# Autodesk Inventor assembly: Eierkocher_final
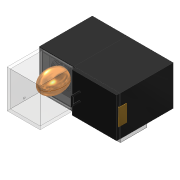
[picture p0: Inventor's stored thumbnail of the model, 180x180]
Saved by Autodesk Inventor 2020 (Build 240168000, 168)
## iProperties
Created: 2022-02-08
Part Number: Eierkocher_final
Document SubType Name: Assembly
Designer: Julian Uhl
Author: Julian Uhl
## Documents named in this file (33)
- C:\Schule\Eier-Inventor\Eierkocher_final.iam
- C:\Schule\Eier-Inventor\Eierkocher_final.ipt
- C:\Schule\Eier-Inventor\EierkocherTeil2.ipt
- C:\Schule\Eier-Inventor\Eihalter_Halter.ipt
- C:\Schule\Eier-Inventor\Raspberry_Dummy.ipt
- C:\Schule\Eier-Inventor\Dichtung_final.ipt
- C:\Schule\Eier-Inventor\Deckel_Koch_final.ipt
- C:\Schule\Eier-Inventor\Eihalter.ipt
- C:\Schule\Eier-Inventor\Ei_groß.ipt
- C:\Schule\Eier-Inventor\Senso_Halter.ipt
- C:\Schule\Eier-Inventor\Display_Dummy.ipt
- C:\Schule\Eier-Inventor\Heiz_Dummy.ipt
- C:\Schule\Eier-Inventor\Wasserbecken.ipt
- C:\Schule\Eier-Inventor\DeckelMess_Better.ipt
- C:\Schule\Eier-Inventor\Schanier1.ipt
- C:\Schule\Eier-Inventor\Schanier2.ipt
- C:\Schule\Eier-Inventor\Schanier3.ipt
- C:\Schule\Eier-Inventor\Ei.ipt
- C:\Schule\Eier-Inventor\Sensor_Dummy.ipt
- C:\Schule\Eier-Inventor\Eierkocher_final\AIP\FEA\dvr005z6o.fins
- C:\Schule\Eier-Inventor\Eierkocher_final\AIP\FEA\dvr005z6o.fsat
- C:\Schule\Eier-Inventor\Eierkocher_final\AIP\FEA\dvr005z6o.ftes
- C:\Schule\Eier-Inventor\Eierkocher_final\AIP\FEA\dvr005z6o.fwiz
- C:\Schule\Eier-Inventor\Eierkocher_final\AIP\FEA\dvr005zeo.fmsh
- C:\Schule\Eier-Inventor\Eierkocher_final\AIP\FEA\dvr005zep.fres
- C:\Schule\Eier-Inventor\Eierkocher_final\AIP\FEA\dvuwvce80.fins
- C:\Schule\Eier-Inventor\Eierkocher_final\AIP\FEA\dvuwvce80.fsat
- C:\Schule\Eier-Inventor\Eierkocher_final\AIP\FEA\dvuwvce80.ftes
- C:\Schule\Eier-Inventor\Eierkocher_final\AIP\FEA\dvuwvce80.fwiz
- C:\Schule\Eier-Inventor\Eierkocher_final\AIP\FEA\dvuwvcekg.fmsh
- C:\Schule\Eier-Inventor\Eierkocher_final\AIP\FEA\dvuwvcekh.fres
- C:\Schule\Eier-Inventor\Eierkocher_final\AIP\FEA\dvyb0c0e8.fmsh
- C:\Schule\Eier-Inventor\Eierkocher_final\AIP\FEA\dvyb0c0e9.fres
## Components (21 placed, 18 different names)
1. Eierkocher_final:1 — Passend:1, Fluchtend:1, Fluchtend:2, Passend:2, Passend:3, Fluchtend:3, Passend:4, Passend:5, Fluchtend:4, Passend:6, Passend:7, Fluchtend:5, Passend:8, Passend:9, Fluchtend:6, Passend:13, Passend:14, Passend:15, Passend:17, Passend:18, Passend:35, Passend:36, Passend:37, Passend:41, Passend:44, Passend:54, Passend:55
2. EierkocherTeil2:1 — Passend:1, Fluchtend:1, Fluchtend:2, Passend:10, Passend:11, Passend:12, Passend:25, Passend:26, Passend:27, Passend:32, Fluchtend:9, Fluchtend:10, Passend:50, Fluchtend:13, Fluchtend:14
3. Eihalter_Halter:1 — Passend:2, Passend:3, Fluchtend:3
4. Eihalter_Halter:2 — Passend:4, Passend:5, Fluchtend:4
5. Eihalter_Halter:3 — Passend:6, Passend:7, Fluchtend:5
6. Eihalter_Halter:4 — Passend:8, Passend:9, Fluchtend:6, Passend:53
7. Raspberry_Dummy:1 — Passend:10, Passend:11, Passend:12
8. Dichtung_final:1 — Passend:13, Passend:14, Passend:15, Passend:16
9. Deckel_Koch_final:1 — Passend:16, Passend:17, Passend:18
10. Senso_Halter:1 — Passend:25, Passend:26, Passend:27, Passend:51, Passend:52, Passend:61, Passend:62, Passend:63
11. Display_Dummy:1 — Passend:32, Fluchtend:9, Fluchtend:10
12. Wasserbecken:1 — Passend:35, Passend:36, Passend:37, Passend:58, Passend:59, Passend:60
13. DeckelMess_Better:1 — Passend:47, Passend:48, Passend:49
14. Schanier1:1 — Passend:45, Fluchtend:11, Passend:47, Passend:48, Passend:49
15. Schanier2:1 — Passend:46, Fluchtend:12, Passend:50, Fluchtend:13, Fluchtend:14
16. Schanier3:1 — Passend:45, Fluchtend:11, Passend:46, Fluchtend:12
17. Ei:1 — Passend:51, Passend:52
18. Eihalter:1 — Passend:53, Passend:54, Passend:55, Passend:56, Passend:57
19. Ei_groß:1 — Passend:56, Passend:57
20. Heiz_Dummy:1 — Passend:58, Passend:59, Passend:60
21. Sensor_Dummy:1 — Passend:61, Passend:62, Passend:63
## Relationships (58: Mate 46, Flush 12)
- Passend:1 [Mate]: Eierkocher_final:1 ↔ EierkocherTeil2:1
- Fluchtend:1 [Flush]: Eierkocher_final:1 ↔ EierkocherTeil2:1
- Fluchtend:2 [Flush]: Eierkocher_final:1 ↔ EierkocherTeil2:1
- Passend:2 [Mate]: Eierkocher_final:1 ↔ Eihalter_Halter:1
- Passend:3 [Mate]: Eierkocher_final:1 ↔ Eihalter_Halter:1
- Fluchtend:3 [Flush] (25 mm): Eierkocher_final:1 ↔ Eihalter_Halter:1
- Passend:4 [Mate]: Eierkocher_final:1 ↔ Eihalter_Halter:2
- Passend:5 [Mate]: Eierkocher_final:1 ↔ Eihalter_Halter:2
- Fluchtend:4 [Flush] (25 mm): Eierkocher_final:1 ↔ Eihalter_Halter:2
- Passend:6 [Mate]: Eierkocher_final:1 ↔ Eihalter_Halter:3
- Passend:7 [Mate]: Eierkocher_final:1 ↔ Eihalter_Halter:3
- Fluchtend:5 [Flush] (25 mm): Eierkocher_final:1 ↔ Eihalter_Halter:3
- Passend:8 [Mate]: Eierkocher_final:1 ↔ Eihalter_Halter:4
- Passend:9 [Mate]: Eierkocher_final:1 ↔ Eihalter_Halter:4
- Fluchtend:6 [Flush] (25 mm): Eierkocher_final:1 ↔ Eihalter_Halter:4
- Passend:10 [Mate]: EierkocherTeil2:1 ↔ Raspberry_Dummy:1
- Passend:11 [Mate] (15 mm): EierkocherTeil2:1 ↔ Raspberry_Dummy:1
- Passend:12 [Mate] (20 mm): EierkocherTeil2:1 ↔ Raspberry_Dummy:1
- Passend:13 [Mate]: Eierkocher_final:1 ↔ Dichtung_final:1
- Passend:14 [Mate] (1 mm): Eierkocher_final:1 ↔ Dichtung_final:1
- Passend:15 [Mate] (1 mm): Eierkocher_final:1 ↔ Dichtung_final:1
- Passend:16 [Mate]: Dichtung_final:1 ↔ Deckel_Koch_final:1
- Passend:17 [Mate]: Eierkocher_final:1 ↔ Deckel_Koch_final:1
- Passend:18 [Mate]: Eierkocher_final:1 ↔ Deckel_Koch_final:1
- Passend:25 [Mate]: EierkocherTeil2:1 ↔ Senso_Halter:1
- Passend:26 [Mate]: EierkocherTeil2:1 ↔ Senso_Halter:1
- Passend:27 [Mate]: EierkocherTeil2:1 ↔ Senso_Halter:1
- Passend:32 [Mate]: EierkocherTeil2:1 ↔ Display_Dummy:1
- Fluchtend:9 [Flush] (5 mm): EierkocherTeil2:1 ↔ Display_Dummy:1
- Fluchtend:10 [Flush] (5 mm): EierkocherTeil2:1 ↔ Display_Dummy:1
- Passend:35 [Mate]: Eierkocher_final:1 ↔ Wasserbecken:1
- Passend:36 [Mate] (5 mm): Eierkocher_final:1 ↔ Wasserbecken:1
- Passend:37 [Mate] (5 mm): Eierkocher_final:1 ↔ Wasserbecken:1
- Passend:41 [Mate]: Eierkocher_final:1
- Passend:44 [Mate]: Eierkocher_final:1
- Passend:45 [Mate]: Schanier1:1 ↔ Schanier3:1
- Fluchtend:11 [Flush]: Schanier1:1 ↔ Schanier3:1
- Passend:46 [Mate]: Schanier2:1 ↔ Schanier3:1
- Fluchtend:12 [Flush]: Schanier2:1 ↔ Schanier3:1
- Passend:47 [Mate]: DeckelMess_Better:1 ↔ Schanier1:1
- Passend:48 [Mate] (3 mm): DeckelMess_Better:1 ↔ Schanier1:1
- Passend:49 [Mate] (2 mm): DeckelMess_Better:1 ↔ Schanier1:1
- Passend:50 [Mate]: EierkocherTeil2:1 ↔ Schanier2:1
- Fluchtend:13 [Flush] (35 mm): EierkocherTeil2:1 ↔ Schanier2:1
- Fluchtend:14 [Flush] (142 mm): EierkocherTeil2:1 ↔ Schanier2:1
- Passend:51 [Mate]: Senso_Halter:1 ↔ Ei:1
- Passend:52 [Mate] (10 mm): Senso_Halter:1 ↔ Ei:1
- Passend:53 [Mate]: Eihalter_Halter:4 ↔ Eihalter:1
- Passend:54 [Mate]: Eierkocher_final:1 ↔ Eihalter:1
- Passend:55 [Mate]: Eierkocher_final:1 ↔ Eihalter:1
- Passend:56 [Mate]: Eihalter:1 ↔ Ei_groß:1
- Passend:57 [Mate] (30 mm): Eihalter:1 ↔ Ei_groß:1
- Passend:58 [Mate] (3.25 mm): Wasserbecken:1 ↔ Heiz_Dummy:1
- Passend:59 [Mate] (10 mm): Wasserbecken:1 ↔ Heiz_Dummy:1
- Passend:60 [Mate] (3.25 mm): Wasserbecken:1 ↔ Heiz_Dummy:1
- Passend:61 [Mate]: Senso_Halter:1 ↔ Sensor_Dummy:1
- Passend:62 [Mate]: Senso_Halter:1 ↔ Sensor_Dummy:1
- Passend:63 [Mate]: Senso_Halter:1 ↔ Sensor_Dummy:1
## Named parameters: sa_0 = 60, sa_2 = -60, sa_3 = 2e-13, sa_4 = -5e-13, sa_1 = 1, sa_5 = 0.6
note: some values were not read from the file. Shown as the stored number, unit unknown: "sa_0", "sa_2", "sa_3", "sa_4", "sa_1", "sa_5".
